# Autodesk Inventor assembly: protectar
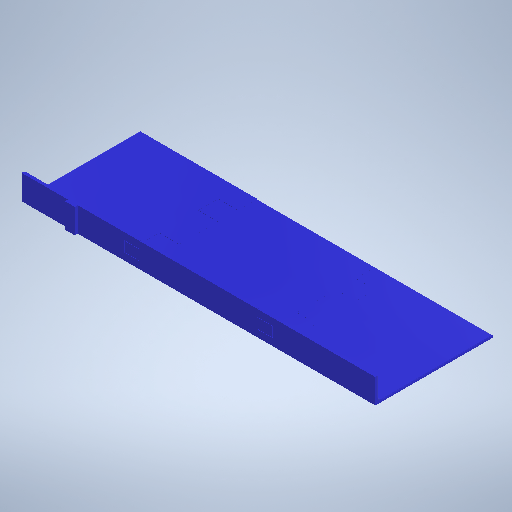
[picture p0: Inventor's stored thumbnail of the model, 512x512]
Saved by Autodesk Inventor 2025 (Build 290162000, 162)
## iProperties
Created: 2025-11-20
Part Number: protectar
Document SubType Name: Assembly
Designer: sooo1
Author: sooo1
## Documents named in this file (5)
- C:\Users\sooo1\Downloads\final-20260216T060151Z-1-001\final\field\protectar.iam
- C:\Users\sooo1\Downloads\final-20260216T060151Z-1-001\final\field\protectar2.ipt
- C:\Users\sooo1\Downloads\final-20260216T060151Z-1-001\final\field\protectar3.ipt
- C:\Users\sooo1\Downloads\final-20260216T060151Z-1-001\final\field\protectar1.ipt
- C:\Users\sooo1\Downloads\final-20260216T060151Z-1-001\final\field\marker.ipt
## Components (4 placed, 4 different names)
1. protectar1:1 — フラッシュ:2, メイト:1, メイト:3
2. protectar2:1 — フラッシュ:1, フラッシュ:2, メイト:1, メイト:2, メイト:3, メイト:4, フラッシュ:3, フラッシュ:4, フラッシュ:5, メイト:5, フラッシュ:6
3. protectar3:1 — フラッシュ:1, メイト:2, メイト:4
4. marker:1 — メイト:5, フラッシュ:6
## Relationships (11: Flush 6, Mate 5)
- フラッシュ:1 [Flush]: protectar2:1 ↔ protectar3:1
- フラッシュ:2 [Flush]: protectar1:1 ↔ protectar2:1
- メイト:1 [Mate]: protectar1:1 ↔ protectar2:1
- メイト:2 [Mate]: protectar2:1 ↔ protectar3:1
- メイト:3 [Mate]: protectar1:1 ↔ protectar2:1
- メイト:4 [Mate]: protectar2:1 ↔ protectar3:1
- フラッシュ:3 [Flush]: protectar2:1
- フラッシュ:4 [Flush]: protectar2:1
- フラッシュ:5 [Flush]: protectar2:1
- メイト:5 [Mate]: protectar2:1 ↔ marker:1
- フラッシュ:6 [Flush]: protectar2:1 ↔ marker:1
